# Autodesk Inventor assembly: バネねじり270.z3
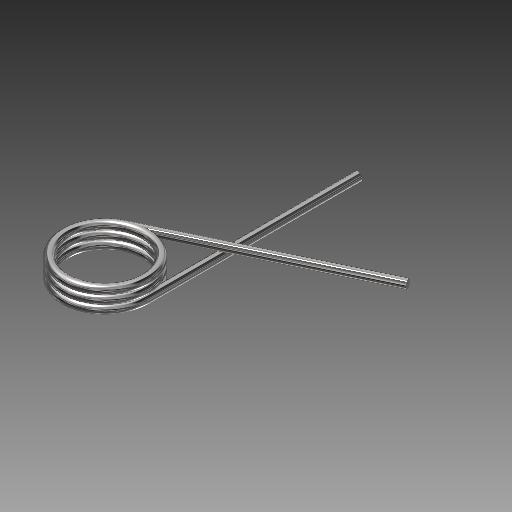
[picture p0: Inventor's stored thumbnail of the model, 512x512]
Saved by Autodesk Inventor 2020 (Build 240168000, 168)
## iProperties
Created: 2018-12-29
Part Number: バネねじり270.z3
Material: 一般
Document SubType Name: Assembly
Designer: 雪村
Mass: 1.42921 g
Surface Area: 6.15825 cm^2
Volume: 0.182065 cm^3
Density: 7.85 g/cm^3
Author: 雪村
## Documents named in this file (3)
- C:\Users\white\Documents\SRDC\SRDC\Inventor_2017\2018年機体\パーツ\バネねじり270.z3.iam
- C:\Users\white\Documents\SRDC\SRDC\Inventor_2017\2018年機体\パーツ\バネねじり270.z3.1.ipt
- C:\Users\white\Documents\SRDC\SRDC\Inventor_2017\2018年機体\パーツ\バネねじり270.z3.2.ipt
## Components (2 placed, 2 different names)
1. バネねじり270.z3.1:1 — 正接:3, 角度:2, メイト:3
2. バネねじり270.z3.2:1 — メイト:3, メイト:4
## Relationships (4: Mate 2, Tangent 1, Angle 1)
- 正接:3 [Tangent]: バネねじり270.z3.1:1
- 角度:2 [Angle] (0 deg): バネねじり270.z3.1:1
- メイト:3 [Mate]: バネねじり270.z3.1:1 ↔ バネねじり270.z3.2:1
- メイト:4 [Mate] (1.8 mm): バネねじり270.z3.2:1
